# Autodesk Inventor assembly: legs_asm_alt
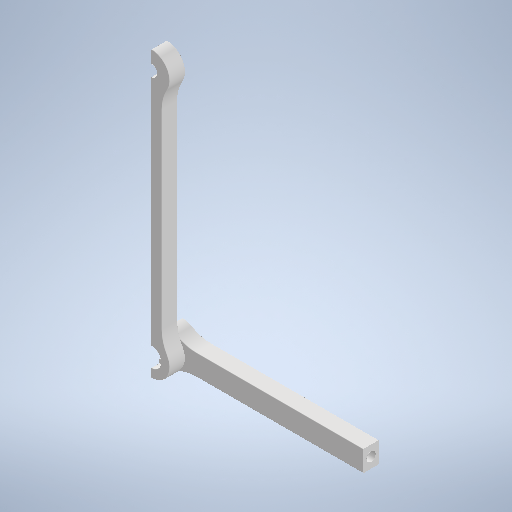
[picture p0: Inventor's stored thumbnail of the model, 512x512]
Saved by Autodesk Inventor 2025.1 (Build 291241000, 241)
## iProperties
Created: 2024-11-08
Part Number: legs_asm_alt
Document SubType Name: Assembly
Designer: ZOMBULLI
Author: ZOMBULLI
## Documents named in this file (3)
- C:\Users\zombulli\OneDrive - Carl Zeiss AG\Desktop\DHBW\Semester 5\mte380\Stewart Platform_new\legs_asm_alt.iam
- C:\Users\zombulli\OneDrive - Carl Zeiss AG\Desktop\DHBW\Semester 5\mte380\Stewart Platform_new\alternativeJoint - Kopie.ipt
- C:\Users\zombulli\OneDrive - Carl Zeiss AG\Desktop\DHBW\Semester 5\mte380\Stewart Platform_new\alternativeJoint2 - Kopie.ipt
## Components (2 placed, 2 different names)
1. alternativeJoint - Kopie:1 — Passend:1, Passend:2, Winkel:1
2. alternativeJoint2 - Kopie:1 — Passend:1, Passend:2, Winkel:1
## Relationships (3: Mate 2, Angle 1)
- Passend:1 [Mate] (0.2 mm): alternativeJoint - Kopie:1 ↔ alternativeJoint2 - Kopie:1
- Passend:2 [Mate]: alternativeJoint - Kopie:1 ↔ alternativeJoint2 - Kopie:1
- Winkel:1 [Angle] (90 deg): alternativeJoint - Kopie:1 ↔ alternativeJoint2 - Kopie:1
